# Autodesk Inventor assembly: Assembly1
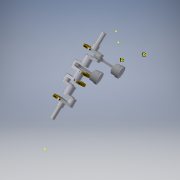
[picture p0: Inventor's stored thumbnail of the model, 180x180]
Saved by Autodesk Inventor 2019 (Build 230136000, 136)
## iProperties
Created: 2019-06-29
Part Number: Assembly1
Document SubType Name: Assembly
Designer: usuario
Mass: 22.4741 g
Surface Area: 125.407 cm^2
Volume: 21.3835 cm^3
Density: 1.051 g/cm^3
Author: usuario
## Documents named in this file (11)
- E:\OSCAR\UNAL\6to SEMESTRE\Principios de dinámica\Proyectos\Proyecto 2\Mio\Sin_Vibraciones.iam
- E:\OSCAR\UNAL\6to SEMESTRE\Principios de dinámica\Proyectos\Proyecto 2\Mio\cigueñal.ipt
- E:\OSCAR\UNAL\6to SEMESTRE\Principios de dinámica\Proyectos\Proyecto 2\Mio\Contrapeso2.ipt
- E:\OSCAR\UNAL\6to SEMESTRE\Principios de dinámica\Proyectos\Proyecto 2\Mio\Contrapeso1.ipt
- E:\OSCAR\UNAL\6to SEMESTRE\Principios de dinámica\Proyectos\Proyecto 2\Mio\Contrapeso4.ipt
- E:\OSCAR\UNAL\6to SEMESTRE\Principios de dinámica\Proyectos\Proyecto 2\Mio\Contrapeso5.ipt
- E:\OSCAR\UNAL\6to SEMESTRE\Principios de dinámica\Proyectos\Proyecto 2\Mio\Pasador 2.ipt
- E:\OSCAR\UNAL\6to SEMESTRE\Principios de dinámica\Proyectos\Proyecto 2\Mio\piston.ipt
- E:\OSCAR\UNAL\6to SEMESTRE\Principios de dinámica\Proyectos\Proyecto 2\Mio\biela1.ipt
- E:\OSCAR\UNAL\6to SEMESTRE\Principios de dinámica\Proyectos\Proyecto 2\Mio\biela2.ipt
- E:\OSCAR\UNAL\6to SEMESTRE\Principios de dinámica\Proyectos\Proyecto 2\Mio\Union.ipt
## Components (20 placed, 10 different names)
1. cigueñal:1 — Rigid:2, Rotational:1, Rotational:2, Rotational:3, Insert:3, Insert:6, Insert:7, Insert:8, Rigid:3, Insert:9, Rotational:6, Rotational:7, Insert:13
2. Contrapeso2:1 — Rigid:2, Insert:4, Insert:5
3. Contrapeso1:1 — Rotational:1, Rotational:7
4. Contrapeso4:1 — Rotational:2, Rigid:3
5. Contrapeso5:1 — Rotational:3, Insert:2, Insert:10, Rotational:6
6. Pasador 2:1 — Insert:3
7. Pasador 2:2 — Insert:4
8. Pasador 2:3 — Insert:10
9. Pasador 2:4 — Insert:2
10. Pasador 2:5 — Insert:8
11. Pasador 2:6 — Insert:7
12. Pasador 2:7 — Insert:5
13. Pasador 2:8 — Insert:6
14. piston:2 — Mate:1, Mate:2
15. biela1:1 — Rotational:4, Rotational:5
16. biela2:1 — Insert:9, Rotational:4, Rotational:5, Insert:11
17. Union:4 — Insert:11, Mate:1, Mate:2
18. piston:5 — Mate:4
19. biela2:5 — Insert:13
20. Union:5 — Mate:4
## Relationships (25: Insert 12, RevoluteJoint 7, Mate 4, WeldJoint 2)
- Rigid:2 [WeldJoint]: cigueñal:1 ↔ Contrapeso2:1
- Rotational:1 [RevoluteJoint]: cigueñal:1 ↔ Contrapeso1:1
- Rotational:2 [RevoluteJoint]: cigueñal:1 ↔ Contrapeso4:1
- Rotational:3 [RevoluteJoint]: cigueñal:1 ↔ Contrapeso5:1
- Insert:2 (-7 mm): Contrapeso5:1 ↔ Pasador 2:4
- Insert:3 (-9 mm): cigueñal:1 ↔ Pasador 2:1
- Insert:4 (-7 mm): Contrapeso2:1 ↔ Pasador 2:2
- Insert:5 (-7 mm): Contrapeso2:1 ↔ Pasador 2:7
- Insert:6 (-9 mm): cigueñal:1 ↔ Pasador 2:8
- Insert:7 (-9 mm): cigueñal:1 ↔ Pasador 2:6
- Insert:8 (-9 mm): cigueñal:1 ↔ Pasador 2:5
- Rigid:3 [WeldJoint]: cigueñal:1 ↔ Contrapeso4:1
- Insert:9 (-0.4 mm): cigueñal:1 ↔ biela2:1
- Rotational:4 [RevoluteJoint]: biela1:1 ↔ biela2:1
- Rotational:5 [RevoluteJoint]: biela1:1 ↔ biela2:1
- Insert:10 (-6 mm): Contrapeso5:1 ↔ Pasador 2:3
- Rotational:6 [RevoluteJoint]: cigueñal:1 ↔ Contrapeso5:1
- Rotational:7 [RevoluteJoint]: cigueñal:1 ↔ Contrapeso1:1
- Insert:11 (-11 mm): biela2:1 ↔ Union:4
- Mate:1: piston:2 ↔ Union:4
- Mate:2: piston:2 ↔ Union:4
- [Insert] (-11 mm): biela2:5 ↔ Union:5
- [Mate]: piston:5 ↔ Union:5
- Insert:13: cigueñal:1 ↔ biela2:5
- Mate:4: piston:5 ↔ Union:5
## Named parameters: d47_d45 = 0 mm, d49_d40 = -11 mm
